# Autodesk Inventor assembly: BuddyRobotASM
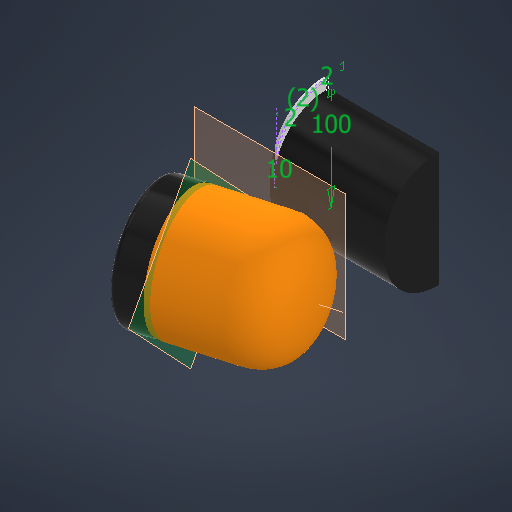
[picture p0: Inventor's stored thumbnail of the model, 512x512]
Saved by Autodesk Inventor 2026.2 (Build 302298000, 298)
## iProperties
Created: 2026-06-05
Part Number: BuddyRobotASM
Document SubType Name: Assembly
Designer: User
Author: User
## Documents named in this file (8)
- C:\Users\User\MyWorkspaces\DesktopBuddyRobot\BuddyRobot3DModel\BuddyRobotASM.iam
- C:\Users\User\MyWorkspaces\DesktopBuddyRobot\BuddyRobot3DModel\DisplayCover.ipt
- C:\Users\User\MyWorkspaces\DesktopBuddyRobot\BuddyRobot3DModel\DisplayGlassDark.ipt
- C:\Users\User\MyWorkspaces\DesktopBuddyRobot\BuddyRobot3DModel\DisplayGlass.ipt
- C:\Users\User\MyWorkspaces\DesktopBuddyRobot\BuddyRobot3DModel\Display\Display\Display.iam
- C:\Users\User\MyWorkspaces\DesktopBuddyRobot\BuddyRobot3DModel\Head.ipt
- C:\Users\User\MyWorkspaces\DesktopBuddyRobot\BuddyRobot3DModel\BuddyRobotBase.ipt
- C:\Users\User\MyWorkspaces\DesktopBuddyRobot\BuddyRobot3DModel\BuddyRobotBaseDoor.ipt
## Components (7 placed, 7 different names)
1. DisplayCover:1 — Mate:1, Insert:1, Insert:2, Mate:4, Mate:5, Insert:3, Insert:4, Mate:6, Mate:7
2. DisplayGlassDark:1 — Mate:1, Insert:1, Insert:2, Mate:2, Mate:3
3. DisplayGlass:1 — Mate:2, Mate:3, Mate:4
4. Display:1 [sub-assembly] — Mate:5, Insert:3, Insert:4
5. Head:1 — Mate:6, Mate:7, Mate:11, Mate:12
6. BuddyRobotBase:1 — Mate:8, Mate:9, Mate:10, Mate:11, Mate:12, Mate:13, Mate:14
7. BuddyRobotBaseDoor:1 — Mate:13, Mate:14
## Relationships (18: Mate 14, Insert 4)
- Mate:1: DisplayCover:1 ↔ DisplayGlassDark:1
- Insert:1: DisplayCover:1 ↔ DisplayGlassDark:1
- Insert:2: DisplayCover:1 ↔ DisplayGlassDark:1
- Mate:2: DisplayGlassDark:1 ↔ DisplayGlass:1
- Mate:3: DisplayGlassDark:1 ↔ DisplayGlass:1
- Mate:4: DisplayCover:1 ↔ DisplayGlass:1
- Mate:5: DisplayCover:1 ↔ Display:1
- Insert:3: DisplayCover:1 ↔ Display:1
- Insert:4: DisplayCover:1 ↔ Display:1
- Mate:6: DisplayCover:1 ↔ Head:1
- Mate:7: DisplayCover:1 ↔ Head:1
- Mate:8: BuddyRobotBase:1
- Mate:9: BuddyRobotBase:1
- Mate:10: BuddyRobotBase:1
- Mate:11: Head:1 ↔ BuddyRobotBase:1
- Mate:12: Head:1 ↔ BuddyRobotBase:1
- Mate:13: BuddyRobotBase:1 ↔ BuddyRobotBaseDoor:1
- Mate:14: BuddyRobotBase:1 ↔ BuddyRobotBaseDoor:1
